# Autodesk Inventor assembly: QUAT HUT
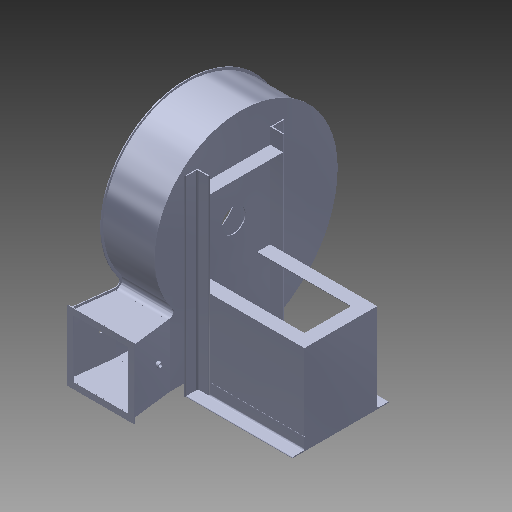
[picture p0: Inventor's stored thumbnail of the model, 512x512]
Saved by Autodesk Inventor 2017 (Build 210142000, 142)
## iProperties
Created: 2013-02-21
Part Number: QUAT HUT
Document SubType Name: Assembly
Designer: XuZhiqing
Sending System: SolidWorks 2013
Last Author: Usr01
Last Saved: 2013-02-23
Author: XuZhiqing
## Documents named in this file (9)
- C:\Users\XuZhiqing\Desktop\Project01-CFD_the_sys\CAD-Whole Sys v1.02\blower\QUAT HUT.iam
- C:\Users\XuZhiqing\Desktop\Project01-CFD_the_sys\CAD-Whole Sys v1.02\blower\KHUNG DO MAY.ipt
- C:\Users\XuZhiqing\Desktop\Project01-CFD_the_sys\CAD-Whole Sys v1.02\blower\MAT TRUOC.ipt
- C:\Users\XuZhiqing\Desktop\Project01-CFD_the_sys\CAD-Whole Sys v1.02\blower\MAT TRUOC_MAT TRUOC.ipt
- C:\Users\XuZhiqing\Desktop\Project01-CFD_the_sys\CAD-Whole Sys v1.02\blower\MAT HONG.ipt
- C:\Users\XuZhiqing\Desktop\Project01-CFD_the_sys\CAD-Whole Sys v1.02\blower\MAT HONG 2.ipt
- C:\Users\XuZhiqing\Desktop\Project01-CFD_the_sys\CAD-Whole Sys v1.02\blower\MAT BICH.iam
- C:\Users\XuZhiqing\Desktop\Project01-CFD_the_sys\CAD-Whole Sys v1.02\blower\LA_3.ipt
- C:\Users\XuZhiqing\Desktop\Project01-CFD_the_sys\CAD-Whole Sys v1.02\blower\CHOT.ipt
## Components (9 placed, 7 different names)
1. KHUNG DO MAY:1
2. MAT TRUOC:1
3. MAT TRUOC:2 — Mate:1, Flush:1
4. MAT HONG:1 — Mate:1
5. MAT HONG 2:1
6. MAT HONG 2:2 — Mate:2, Flush:2
7. MAT BICH:1 [sub-assembly] — Mate:2, Flush:1, Flush:2
8. LA:1
9. CHOT:2
## Relationships (4: Mate 2, Flush 2)
- Mate:1: MAT TRUOC:2 ↔ MAT HONG:1
- Mate:2: MAT HONG 2:2 ↔ MAT BICH:1
- Flush:1: MAT TRUOC:2 ↔ MAT BICH:1
- Flush:2: MAT HONG 2:2 ↔ MAT BICH:1
